# Autodesk Inventor assembly: NEO_550_w_spacer_gt2_pinion
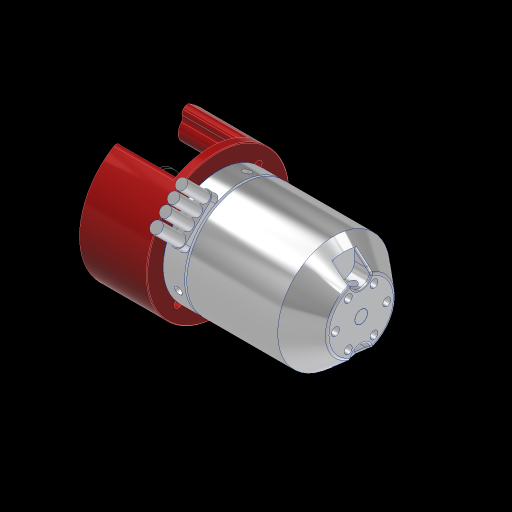
[picture p0: Inventor's stored thumbnail of the model, 512x512]
Saved by Autodesk Inventor 2023.3 (Build 273359000, 359)
## iProperties
Created: 2024-01-20
Part Number: NEO_550_w_spacer_gt2_pinion
Document SubType Name: Assembly
Designer: mavericks
Mass: 145.094 g
Surface Area: 100.941 cm^2
Volume: 41.0259 cm^3
Density: 3.53663 g/cm^3
Author: mavericks
## Documents named in this file (4)
- C:\Users\mavericks\Desktop\Crescendo_2024-CAD\2024 Robot\COMMON PARTS\MOTORS\NEO_550_w_spacer_gt2_pinion.iam
- C:\Users\mavericks\Desktop\Crescendo_2024-CAD\2024 Robot\COMMON PARTS\MOTORS\REV-21-1651.ipt
- C:\Users\mavericks\Desktop\Crescendo_2024-CAD\2024 Robot\COMMON PARTS\MOTORS\REV-21-1908.ipt
- C:\Users\mavericks\Desktop\Crescendo_2024-CAD\2024 Robot\COMMON PARTS\MOTORS\Neo_550_Spacer.ipt
## Components (3 placed, 3 different names)
1. REV-21-1651:1 — Insert:3, Mate:1, Insert:4, Mate:2
2. REV-21-1908:1 — Insert:3
3. Neo_550_Spacer:1 — Mate:1, Insert:4, Mate:2
## Relationships (4: Insert 2, Mate 2)
- Insert:3: REV-21-1651:1 ↔ REV-21-1908:1
- Mate:1: REV-21-1651:1 ↔ Neo_550_Spacer:1
- Insert:4: REV-21-1651:1 ↔ Neo_550_Spacer:1
- Mate:2: REV-21-1651:1 ↔ Neo_550_Spacer:1
